# Autodesk Inventor assembly: 10-J1_new
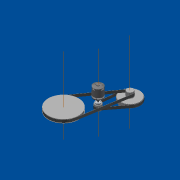
[picture p0: Inventor's stored thumbnail of the model, 180x180]
Saved by Autodesk Inventor 2018 (Build 220112000, 112)
## iProperties
Created: 2020-07-27
Part Number: 10-J1_new
Document SubType Name: Assembly
Designer: Bunny320
Author: Bunny320
## Documents named in this file (5)
- C:\Users\Bunny320\Desktop\sechs\4-CAD\10-J1_new.iam
- C:\Users\Bunny320\Desktop\sechs\4-CAD\generated\J1_belts_lower.iam
- C:\Users\Bunny320\Desktop\sechs\4-CAD\generated\J1_belts_upper.iam
- C:\Users\Bunny320\Desktop\sechs\4-CAD\standardParts\Pololu mounting hub\pololu-universal-aluminum-mounting-hub-for-5mm-shaft-m3-holes.ipt
- C:\Users\Bunny320\Desktop\sechs\4-CAD\standardParts\AS 2820 kv880\AS 2820 kv880.ipt
## Components (4 placed, 4 different names)
1. J1_belts_lower:1 [sub-assembly] — Mate:1, Flush:1, Flush:2, Flush:3, Mate:2, Mate:3, Mate:5
2. J1_belts_upper:1 [sub-assembly] — Mate:1, Mate:2
3. pololu-universal-aluminum-mounting-hub-for-5mm-shaft-m3-holes:1 — Mate:3, Flush:4, Mate:4, Mate:5
4. AS 2820 kv880:1 — Flush:4, Mate:4
## Relationships (9: Mate 5, Flush 4)
- Mate:1: J1_belts_lower:1 ↔ J1_belts_upper:1
- Flush:1: J1_belts_lower:1
- Flush:2: J1_belts_lower:1
- Flush:3: J1_belts_lower:1
- Mate:2: J1_belts_lower:1 ↔ J1_belts_upper:1
- Mate:3: J1_belts_lower:1 ↔ pololu-universal-aluminum-mounting-hub-for-5mm-shaft-m3-holes:1
- Flush:4: pololu-universal-aluminum-mounting-hub-for-5mm-shaft-m3-holes:1 ↔ AS 2820 kv880:1
- Mate:4: pololu-universal-aluminum-mounting-hub-for-5mm-shaft-m3-holes:1 ↔ AS 2820 kv880:1
- Mate:5: J1_belts_lower:1 ↔ pololu-universal-aluminum-mounting-hub-for-5mm-shaft-m3-holes:1
